# Autodesk Inventor assembly: Kauri Assembly
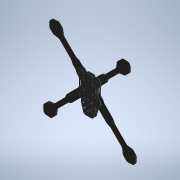
[picture p0: Inventor's stored thumbnail of the model, 180x180]
Saved by Autodesk Inventor 2020 (Build 240168000, 168)
## iProperties
Created: 2022-08-09
Part Number: Kauri Assembly
Document SubType Name: Assembly
Designer: Steven
Author: Steven
## Documents named in this file (5)
- Y:\FPV drone stuff\0 Street League\Frames\PB-Kauri-X\3D prints\35 mm canopy\work in progress prints\Canopy mods\Kauri Assembly.iam
- Y:\FPV drone stuff\0 Street League\Frames\PB-Kauri-X\Kauri bottom plate.ipt
- Y:\FPV drone stuff\0 Street League\Frames\PB-Kauri-X\Kauri mid plate v2.ipt
- Y:\FPV drone stuff\0 Street League\Frames\experimental-quad-frames\modified Kauri arms\disc aero arms\Kauri arm disc aero.ipt
- Y:\FPV drone stuff\0 Street League\Frames\experimental-quad-frames\modified Kauri arms\disc aero arms\Kauri arm long disc aero.ipt
## Components (6 placed, 4 different names)
1. Kauri bottom plate:1 — Mate:1, Mate:2, Flush:1, Flush:2, Flush:3, Mate:3, Mate:4, Mate:5, Mate:6, Mate:7, Mate:8, Mate:9, Mate:10, Mate:11, Mate:12
2. Kauri mid plate v2:1 — Mate:13, Mate:14, Mate:15
3. Kauri arm disc aero:1 — Mate:1, Mate:3, Mate:5
4. Kauri arm disc aero:2 — Mate:2, Mate:4, Mate:6, Mate:14, Mate:15
5. Kauri arm long disc aero:1 — Mate:8, Mate:10, Mate:11
6. Kauri arm long disc aero:2 — Mate:7, Mate:9, Mate:12, Mate:13
## Relationships (18: Mate 15, Flush 3)
- Mate:1: Kauri bottom plate:1 ↔ Kauri arm disc aero:1
- Mate:2: Kauri bottom plate:1 ↔ Kauri arm disc aero:2
- Flush:1: Kauri bottom plate:1
- Flush:2: Kauri bottom plate:1
- Flush:3: Kauri bottom plate:1
- Mate:3: Kauri bottom plate:1 ↔ Kauri arm disc aero:1
- Mate:4: Kauri bottom plate:1 ↔ Kauri arm disc aero:2
- Mate:5: Kauri bottom plate:1 ↔ Kauri arm disc aero:1
- Mate:6: Kauri bottom plate:1 ↔ Kauri arm disc aero:2
- Mate:7: Kauri bottom plate:1 ↔ Kauri arm long disc aero:2
- Mate:8: Kauri bottom plate:1 ↔ Kauri arm long disc aero:1
- Mate:9: Kauri bottom plate:1 ↔ Kauri arm long disc aero:2
- Mate:10: Kauri bottom plate:1 ↔ Kauri arm long disc aero:1
- Mate:11: Kauri bottom plate:1 ↔ Kauri arm long disc aero:1
- Mate:12: Kauri bottom plate:1 ↔ Kauri arm long disc aero:2
- Mate:13: Kauri mid plate v2:1 ↔ Kauri arm long disc aero:2
- Mate:14: Kauri mid plate v2:1 ↔ Kauri arm disc aero:2
- Mate:15: Kauri mid plate v2:1 ↔ Kauri arm disc aero:2
